# Autodesk Inventor assembly: upper_shell
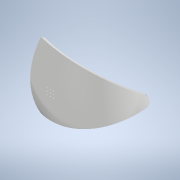
[picture p0: Inventor's stored thumbnail of the model, 180x180]
Saved by Autodesk Inventor 2020.2 (Build 242310000, 310)
## iProperties
Created: 2020-11-22
Part Number: upper_shell
Document SubType Name: Assembly
Designer: mazzo
Author: mazzo
## Documents named in this file (3)
- D:\Documenti\università\Progetto Meccanica dei Robot\assembled in urdf\upper_shell.iam
- D:\Documenti\università\Progetto Meccanica dei Robot\meccanica\parti autodesk\V6\V6 Luca\Motore2.ipt
- D:\Documenti\università\Progetto Meccanica dei Robot\meccanica\parti autodesk\V6\V6 Luca\upper_shell.ipt
## Components (2 placed, 2 different names)
1. Motore2:1 — Coincidente:1, Coincidente:2, Angolo:1, Coincidente:3, Coincidente:4, Coincidente:5
2. upper_shell:1 — Coincidente:3, Coincidente:4, Coincidente:5
## Relationships (6: Mate 5, Angle 1)
- Coincidente:1 [Mate]: Motore2:1
- Coincidente:2 [Mate]: Motore2:1
- Angolo:1 [Angle] (0 deg): Motore2:1
- Coincidente:3 [Mate]: Motore2:1 ↔ upper_shell:1
- Coincidente:4 [Mate]: Motore2:1 ↔ upper_shell:1
- Coincidente:5 [Mate]: Motore2:1 ↔ upper_shell:1
